# Autodesk Inventor assembly: microb_connection
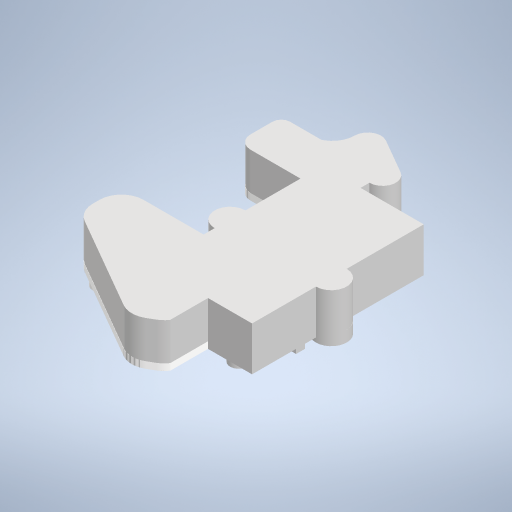
[picture p0: Inventor's stored thumbnail of the model, 512x512]
Saved by Autodesk Inventor 2024.1 (Build 281209000, 209)
## iProperties
Created: 2025-06-17
Part Number: microb_connection
Document SubType Name: Assembly
Designer: hibik
Author: hibik
## Documents named in this file (5)
- C:\Users\hibik\Documents\Robomech\RESCUE\ORCA\hard\board\CORE\microb_connection.iam
- C:\Users\hibik\Documents\Robomech\RESCUE\ORCA\hard\board\CORE\type_A_ver2.ipt
- C:\Users\hibik\Documents\Robomech\RESCUE\ORCA\hard\board\CORE\CORE_hat_outline_typeB_base_ver2.ipt
- C:\Users\hibik\Documents\Robomech\RESCUE\ORCA\hard\board\CORE\CORE_hat_outline_typeB_ver2.ipt
- C:\Users\hibik\Documents\Robomech\RESCUE\ORCA\hard\board\CORE\microb_connection_base.ipt
## Components (4 placed, 4 different names)
1. type_A_ver2:1 — フラッシュ:1, メイト:1, メイト:2, メイト:3, メイト:4
2. CORE_hat_outline_typeB_base_ver2:1 — フラッシュ:1, フラッシュ:2, メイト:1, メイト:2
3. CORE_hat_outline_typeB_ver2:1 — フラッシュ:2, メイト:3, メイト:4
4. microb_connection_base:1 — フラッシュ:3, フラッシュ:4, フラッシュ:5
## Relationships (9: Flush 5, Mate 4)
- フラッシュ:1 [Flush]: type_A_ver2:1 ↔ CORE_hat_outline_typeB_base_ver2:1
- フラッシュ:2 [Flush]: CORE_hat_outline_typeB_base_ver2:1 ↔ CORE_hat_outline_typeB_ver2:1
- メイト:1 [Mate]: type_A_ver2:1 ↔ CORE_hat_outline_typeB_base_ver2:1
- メイト:2 [Mate]: type_A_ver2:1 ↔ CORE_hat_outline_typeB_base_ver2:1
- メイト:3 [Mate]: type_A_ver2:1 ↔ CORE_hat_outline_typeB_ver2:1
- メイト:4 [Mate]: type_A_ver2:1 ↔ CORE_hat_outline_typeB_ver2:1
- フラッシュ:3 [Flush]: microb_connection_base:1
- フラッシュ:4 [Flush]: microb_connection_base:1
- フラッシュ:5 [Flush]: microb_connection_base:1
